# Autodesk Inventor assembly: Frez No,1
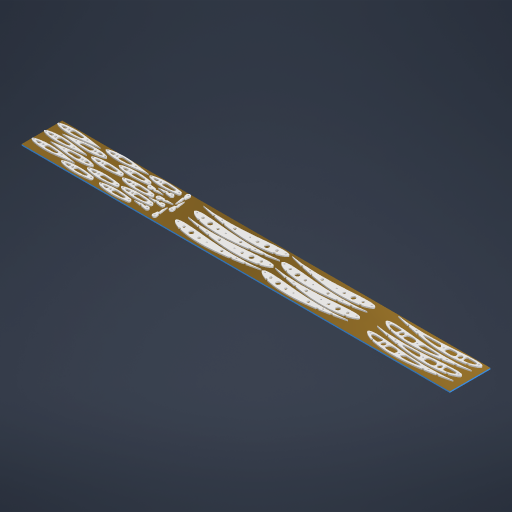
[picture p0: Inventor's stored thumbnail of the model, 512x512]
Saved by Autodesk Inventor 2023 (Build 270158000, 158)
## iProperties
Created: 2023-04-30
Part Number: Frez No,1
Document SubType Name: Assembly
Designer: szykr
Author: szykr
## Documents named in this file (7)
- D:\Folder Instalacyjny\GitHub Pliki\Solaris\new model\Frez_zebra\Frez No,1.iam
- D:\Folder Instalacyjny\GitHub Pliki\Solaris\new model\Frez_zebra\Balsa(95x1000x3).ipt
- D:\Folder Instalacyjny\GitHub Pliki\Solaris\new model\Tail\Tżebro default.ipt
- D:\Folder Instalacyjny\GitHub Pliki\Solaris\new model\Tail\Tżebro z lotkąt.ipt
- D:\Folder Instalacyjny\GitHub Pliki\Solaris\new model\Tail\Tlotka.ipt
- D:\Folder Instalacyjny\GitHub Pliki\Solaris\new model\Żerbo montaż.ipt
- D:\Folder Instalacyjny\GitHub Pliki\Solaris\new model\Żebro default.ipt
## Components (35 placed, 6 different names)
1. Balsa(95x1000x3):1 — Mate:1, Mate:2, Mate:3, Mate:4, Mate:5, Mate:6, Mate:7, Mate:8, Mate:9, Mate:10, Mate:11, Mate:12, Mate:13, Mate:14, Mate:15, Mate:16, Mate:17, Mate:18, Mate:19, Mate:20, Mate:21, Mate:22, Mate:23, Flush:28, Mate:25, Flush:27, Mate:27, Mate:28, Flush:30, Flush:31, Mate:29, Mate:30, Mate:31, Mate:32
2. Tżebro default:1 — Mate:6
3. Tżebro default:2 — Mate:5
4. Tżebro default:3 — Mate:4
5. Tżebro default:4 — Mate:3
6. Tżebro default:5 — Mate:2
7. Tżebro default:6 — Mate:1
8. Tżebro z lotkąt:1 — Mate:14
9. Tżebro z lotkąt:2 — Mate:13
10. Tżebro z lotkąt:3 — Mate:12
11. Tżebro z lotkąt:4 — Mate:11
12. Tżebro z lotkąt:5 — Mate:10
13. Tżebro z lotkąt:6 — Mate:9
14. Tżebro z lotkąt:7 — Mate:8
15. Tżebro z lotkąt:8 — Mate:7
16. Tlotka:1 — Mate:22
17. Tlotka:2 — Mate:21
18. Tlotka:3 — Mate:20
19. Tlotka:4 — Mate:19
20. Tlotka:5 — Mate:18
21. Tlotka:6 — Mate:17
22. Tlotka:7 — Mate:16
23. Tlotka:8 — Mate:15
24. Żerbo montaż:1 — Mate:23
25. Żerbo montaż:2 — Mate:27
26. Żerbo montaż:3 — Mate:25
27. Żerbo montaż:4 — Flush:28
28. Żerbo montaż:5 — Flush:27
29. Żerbo montaż:6 — Mate:28
30. Żerbo montaż:7 — Flush:30
31. Żerbo montaż:8 — Flush:31
32. Żebro default:1 — Mate:32
33. Żebro default:2 — Mate:31
34. Żebro default:3 — Mate:30
35. Żebro default:4 — Mate:29
## Relationships (34: Mate 30, Flush 4)
- Mate:1: Balsa(95x1000x3):1 ↔ Tżebro default:6
- Mate:2: Balsa(95x1000x3):1 ↔ Tżebro default:5
- Mate:3: Balsa(95x1000x3):1 ↔ Tżebro default:4
- Mate:4: Balsa(95x1000x3):1 ↔ Tżebro default:3
- Mate:5: Balsa(95x1000x3):1 ↔ Tżebro default:2
- Mate:6: Balsa(95x1000x3):1 ↔ Tżebro default:1
- Mate:7: Balsa(95x1000x3):1 ↔ Tżebro z lotkąt:8
- Mate:8: Balsa(95x1000x3):1 ↔ Tżebro z lotkąt:7
- Mate:9: Balsa(95x1000x3):1 ↔ Tżebro z lotkąt:6
- Mate:10: Balsa(95x1000x3):1 ↔ Tżebro z lotkąt:5
- Mate:11: Balsa(95x1000x3):1 ↔ Tżebro z lotkąt:4
- Mate:12: Balsa(95x1000x3):1 ↔ Tżebro z lotkąt:3
- Mate:13: Balsa(95x1000x3):1 ↔ Tżebro z lotkąt:2
- Mate:14: Balsa(95x1000x3):1 ↔ Tżebro z lotkąt:1
- Mate:15: Balsa(95x1000x3):1 ↔ Tlotka:8
- Mate:16: Balsa(95x1000x3):1 ↔ Tlotka:7
- Mate:17: Balsa(95x1000x3):1 ↔ Tlotka:6
- Mate:18: Balsa(95x1000x3):1 ↔ Tlotka:5
- Mate:19: Balsa(95x1000x3):1 ↔ Tlotka:4
- Mate:20: Balsa(95x1000x3):1 ↔ Tlotka:3
- Mate:21: Balsa(95x1000x3):1 ↔ Tlotka:2
- Mate:22: Balsa(95x1000x3):1 ↔ Tlotka:1
- Mate:23: Balsa(95x1000x3):1 ↔ Żerbo montaż:1
- Flush:28 (-3 mm): Balsa(95x1000x3):1 ↔ Żerbo montaż:4
- Mate:25: Balsa(95x1000x3):1 ↔ Żerbo montaż:3
- Flush:27 (-3 mm): Balsa(95x1000x3):1 ↔ Żerbo montaż:5
- Mate:27: Balsa(95x1000x3):1 ↔ Żerbo montaż:2
- Mate:28: Balsa(95x1000x3):1 ↔ Żerbo montaż:6
- Flush:30 (-3 mm): Balsa(95x1000x3):1 ↔ Żerbo montaż:7
- Flush:31 (-3 mm): Balsa(95x1000x3):1 ↔ Żerbo montaż:8
- Mate:29: Balsa(95x1000x3):1 ↔ Żebro default:4
- Mate:30: Balsa(95x1000x3):1 ↔ Żebro default:3
- Mate:31: Balsa(95x1000x3):1 ↔ Żebro default:2
- Mate:32: Balsa(95x1000x3):1 ↔ Żebro default:1
